# Autodesk Inventor assembly: Tray Elevator
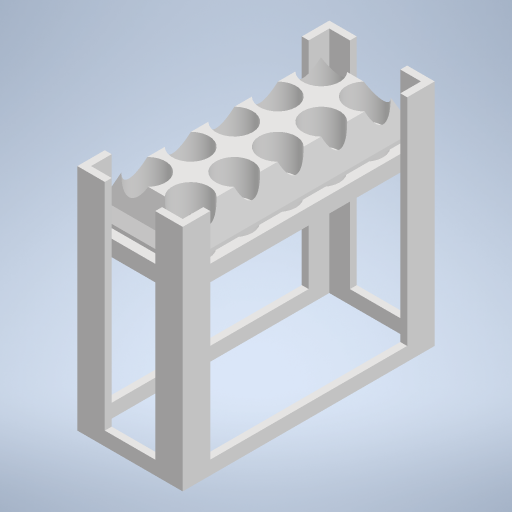
[picture p0: Inventor's stored thumbnail of the model, 512x512]
Saved by Autodesk Inventor 2023 (Build 270158000, 158)
## iProperties
Created: 2023-01-16
Part Number: Tray Elevator
Document SubType Name: Assembly
Designer: Steven
Author: Steven
## Documents named in this file (6)
- C:\Users\steve\OneDrive\Documents\McMaster University\Courses-Year5\4TB6 Capstone Design Project\The_Nursery_Project\parts\Tray Elevator.iam
- C:\Users\steve\OneDrive\Documents\McMaster University\Courses-Year5\4TB6 Capstone Design Project\The_Nursery_Project\parts\frame.ipt
- C:\Users\steve\OneDrive\Documents\McMaster University\Courses-Year5\4TB6 Capstone Design Project\The_Nursery_Project\parts\frame_support.ipt
- C:\Users\steve\OneDrive\Documents\McMaster University\Courses-Year5\4TB6 Capstone Design Project\The_Nursery_Project\parts\frame_support2.ipt
- C:\Users\steve\OneDrive\Documents\McMaster University\Courses-Year5\4TB6 Capstone Design Project\The_Nursery_Project\parts\platform.ipt
- C:\Users\steve\OneDrive\Documents\McMaster University\Courses-Year5\4TB6 Capstone Design Project\The_Nursery_Project\parts\tray.ipt
## Components (10 placed, 5 different names)
1. frame:1 — Mate:1, Flush:3, Flush:4, Mate:6, Flush:11, Flush:12
2. frame:2 — Mate:2, Flush:1, Flush:2, Mate:8, Mate:11
3. frame:3 — Mate:4, Flush:7, Flush:8, Mate:7, Flush:13, Flush:14
4. frame:4 — Mate:3, Flush:5, Flush:6, Mate:5, Flush:9, Flush:10, Mate:9
5. frame_support:1 — Mate:1, Mate:2, Flush:1, Flush:2, Flush:3, Flush:4
6. frame_support:2 — Mate:3, Flush:5, Flush:6, Mate:4, Flush:7, Flush:8
7. frame_support2:1 — Mate:5, Flush:9, Flush:10, Mate:6, Flush:11, Flush:12
8. frame_support2:2 — Mate:7, Flush:13, Flush:14, Mate:11
9. platform:1 — Mate:8, Mate:9, Mate:10, Flush:15, Flush:16
10. tray:1 — Mate:10, Flush:15, Flush:16
## Relationships (27: Flush 16, Mate 11)
- Mate:1: frame:1 ↔ frame_support:1
- Mate:2: frame:2 ↔ frame_support:1
- Flush:1: frame:2 ↔ frame_support:1
- Flush:2: frame:2 ↔ frame_support:1
- Flush:3: frame:1 ↔ frame_support:1
- Flush:4: frame:1 ↔ frame_support:1
- Mate:3: frame:4 ↔ frame_support:2
- Flush:5: frame:4 ↔ frame_support:2
- Flush:6: frame:4 ↔ frame_support:2
- Mate:4: frame:3 ↔ frame_support:2
- Flush:7: frame:3 ↔ frame_support:2
- Flush:8: frame:3 ↔ frame_support:2
- Mate:5: frame:4 ↔ frame_support2:1
- Flush:9: frame:4 ↔ frame_support2:1
- Flush:10: frame:4 ↔ frame_support2:1
- Mate:6: frame:1 ↔ frame_support2:1
- Flush:11: frame:1 ↔ frame_support2:1
- Flush:12: frame:1 ↔ frame_support2:1
- Mate:7: frame:3 ↔ frame_support2:2
- Flush:13: frame:3 ↔ frame_support2:2
- Flush:14: frame:3 ↔ frame_support2:2
- Mate:8: frame:2 ↔ platform:1
- Mate:9: frame:4 ↔ platform:1
- Mate:10: platform:1 ↔ tray:1
- Flush:15: platform:1 ↔ tray:1
- Flush:16: platform:1 ↔ tray:1
- Mate:11: frame:2 ↔ frame_support2:2
